# Autodesk Inventor assembly: THz Rotator Mount Assembly
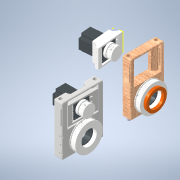
[picture p0: Inventor's stored thumbnail of the model, 180x180]
Saved by Autodesk Inventor 2020 (Build 240168000, 168)
## iProperties
Created: 2024-01-28
Part Number: THz Rotator Mount Assembly
Document SubType Name: Assembly
Designer: Scott
Author: Scott
## Documents named in this file (11)
- C:\Users\Scott\Documents\Inventor\THz Rotator Mount\THz Rotator Mount Assembly.iam
- C:\Users\Scott\Documents\Inventor\THz Rotator Mount\StepperOnline Nema 23 Stepper Motor.ipt
- C:\Users\Scott\Documents\Inventor\THz Rotator Mount\ThorLabs LCRM2_M.ipt
- C:\Users\Scott\Documents\Inventor\THz Rotator Mount\THz Polarizer.ipt
- C:\Users\Scott\Documents\Inventor\THz Rotator Mount\Rotator Mount Base.ipt
- C:\Users\Scott\Documents\Inventor\THz Rotator Mount\Stepper Motor Mount.ipt
- C:\Users\Scott\Documents\Inventor\THz Rotator Mount\Motor Gear Attachment.ipt
- C:\Users\Scott\Documents\Inventor\THz Rotator Mount\THz Polarizer Gear Actuator.ipt
- C:\Users\Scott\Documents\Inventor\THz Rotator Mount\Optical Post.ipt
- C:\Users\Scott\Documents\Inventor\THz Rotator Mount\Stepper Motor Mount v2.0.ipt
- C:\Users\Scott\Documents\Inventor\THz Rotator Mount\Rotator Mount Base v2.0.ipt
## Components (15 placed, 10 different names)
1. StepperOnline Nema 23 Stepper Motor:1 — Mate:2, Mate:6, Mate:7, Insert:1
2. ThorLabs LCRM2_M:1 — Flush:1, Mate:10, Mate:11, Insert:2
3. THz Polarizer:1 — Insert:3, Insert:4
4. Rotator Mount Base:1 — Mate:9, Flush:1, Mate:10, Mate:11, Mate:12, Insert:5, Insert:6, Mate:13, Flush:2, Flush:3
5. Stepper Motor Mount:1 — Mate:2, Mate:6, Mate:7, Mate:9, Mate:12, Mate:13
6. Motor Gear Attachment:1 — Insert:1
7. THz Polarizer Gear Actuator:1 — Insert:2, Insert:3, Insert:4
8. Optical Post:1 — Insert:5
9. Optical Post:2 — Insert:6
10. Stepper Motor Mount v2.0:1 — Mate:14, Mate:15, Mate:16, Mate:19, Mate:20, Mate:21
11. Rotator Mount Base v2.0:1 — Flush:2, Flush:3, Mate:14, Mate:15, Mate:16, Mate:17, Mate:18, Flush:4
12. ThorLabs LCRM2_M:2 — Mate:17, Mate:18, Flush:4, Insert:7
13. THz Polarizer Gear Actuator:2 — Insert:7
14. StepperOnline Nema 23 Stepper Motor:2 — Mate:19, Mate:20, Mate:21, Insert:8
15. Motor Gear Attachment:2 — Insert:8
## Relationships (28: Mate 16, Insert 8, Flush 4)
- Mate:2: StepperOnline Nema 23 Stepper Motor:1 ↔ Stepper Motor Mount:1
- Mate:6: StepperOnline Nema 23 Stepper Motor:1 ↔ Stepper Motor Mount:1
- Mate:7: StepperOnline Nema 23 Stepper Motor:1 ↔ Stepper Motor Mount:1
- Mate:9: Rotator Mount Base:1 ↔ Stepper Motor Mount:1
- Flush:1: ThorLabs LCRM2_M:1 ↔ Rotator Mount Base:1
- Mate:10: ThorLabs LCRM2_M:1 ↔ Rotator Mount Base:1
- Mate:11: ThorLabs LCRM2_M:1 ↔ Rotator Mount Base:1
- Mate:12: Rotator Mount Base:1 ↔ Stepper Motor Mount:1
- Insert:1: StepperOnline Nema 23 Stepper Motor:1 ↔ Motor Gear Attachment:1
- Insert:2 (12.7 mm): ThorLabs LCRM2_M:1 ↔ THz Polarizer Gear Actuator:1
- Insert:3: THz Polarizer:1 ↔ THz Polarizer Gear Actuator:1
- Insert:4: THz Polarizer:1 ↔ THz Polarizer Gear Actuator:1
- Insert:5 (-10 mm): Rotator Mount Base:1 ↔ Optical Post:1
- Insert:6 (-10 mm): Rotator Mount Base:1 ↔ Optical Post:2
- Mate:13 (6 mm): Rotator Mount Base:1 ↔ Stepper Motor Mount:1
- Flush:2: Rotator Mount Base:1 ↔ Rotator Mount Base v2.0:1
- Flush:3: Rotator Mount Base:1 ↔ Rotator Mount Base v2.0:1
- Mate:14 (0.5 mm): Stepper Motor Mount v2.0:1 ↔ Rotator Mount Base v2.0:1
- Mate:15 (0.5 mm): Stepper Motor Mount v2.0:1 ↔ Rotator Mount Base v2.0:1
- Mate:16: Stepper Motor Mount v2.0:1 ↔ Rotator Mount Base v2.0:1
- Mate:17 (0.15 mm): Rotator Mount Base v2.0:1 ↔ ThorLabs LCRM2_M:2
- Mate:18 (0.15 mm): Rotator Mount Base v2.0:1 ↔ ThorLabs LCRM2_M:2
- Flush:4: Rotator Mount Base v2.0:1 ↔ ThorLabs LCRM2_M:2
- Insert:7: ThorLabs LCRM2_M:2 ↔ THz Polarizer Gear Actuator:2
- Mate:19: Stepper Motor Mount v2.0:1 ↔ StepperOnline Nema 23 Stepper Motor:2
- Mate:20: Stepper Motor Mount v2.0:1 ↔ StepperOnline Nema 23 Stepper Motor:2
- Mate:21: Stepper Motor Mount v2.0:1 ↔ StepperOnline Nema 23 Stepper Motor:2
- Insert:8: StepperOnline Nema 23 Stepper Motor:2 ↔ Motor Gear Attachment:2
